# Autodesk Inventor assembly: TF-LC02 (Laser senzor) s
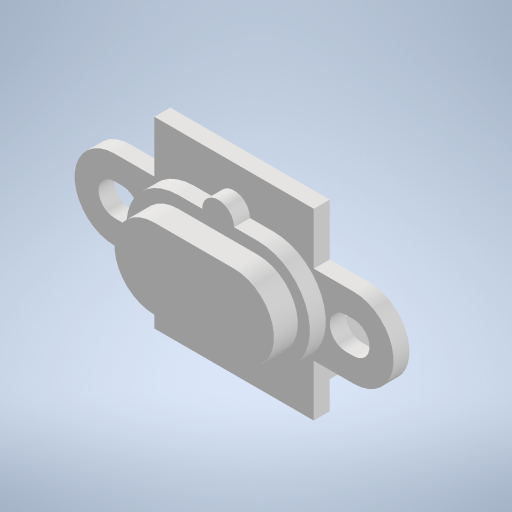
[picture p0: Inventor's stored thumbnail of the model, 512x512]
Saved by Autodesk Inventor 2024 (Build 280153000, 153)
## iProperties
Created: 2023-10-20
Part Number: TF-LC02 (Laser senzor) s
Document SubType Name: Assembly
Designer: jaryj
Author: jaryj
## Documents named in this file (3)
- C:\Users\jaryj\Desktop\Škola\Mini sumo\RoboCop\- 3D -\wip\TF-LC02 (Laser senzor) s.iam
- C:\Users\jaryj\Desktop\Škola\Mini sumo\RoboCop\- 3D -\wip\jst - 1 mm 6 pin female.ipt
- C:\Users\jaryj\Desktop\Škola\Mini sumo\RoboCop\- 3D -\wip\TF-LC02 (Laser senzor).ipt
## Components (2 placed, 2 different names)
1. jst - 1 mm 6 pin female:1 — Proti sobě:1, Stejný směr:1, Stejný směr:2
2. TF-LC02 (Laser senzor):1 — Proti sobě:1, Stejný směr:1, Stejný směr:2
## Relationships (3: Flush 2, Mate 1)
- Proti sobě:1 [Mate]: jst - 1 mm 6 pin female:1 ↔ TF-LC02 (Laser senzor):1
- Stejný směr:1 [Flush] (0.75 mm): jst - 1 mm 6 pin female:1 ↔ TF-LC02 (Laser senzor):1
- Stejný směr:2 [Flush] (1 mm): jst - 1 mm 6 pin female:1 ↔ TF-LC02 (Laser senzor):1
